# Autodesk Inventor assembly: sparIntermediateFlat_US
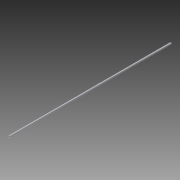
[picture p0: Inventor's stored thumbnail of the model, 180x180]
Saved by Autodesk Inventor 2014 (Build 180170000, 170)
## iProperties
Created: 2015-03-27
Part Number: sparIntermediateFlat_US
Document SubType Name: Assembly
Designer: ddeboer
Author: ddeboer
## Documents named in this file (4)
- C:\Users\ddeboer\Desktop\hera-cad\surface\sparIntermediateFlat_US.iam
- C:\Users\ddeboer\Desktop\hera-cad\surface\pvcSection_2in.ipt
- C:\Users\ddeboer\Desktop\hera-cad\smallParts\coupler_2in.ipt
- C:\Users\ddeboer\Desktop\hera-cad\surface\pvcSection_2in_cut4intermed.ipt
## Components (3 placed, 3 different names)
1. pvcSection_2in:1 — Insert:1
2. coupler_2in:1 — Insert:1, Insert:2
3. pvcSection_2in_cut4intermed:1 — Insert:2
## Relationships (2: Insert 2)
- Insert:1 (-29.3624 mm): pvcSection_2in:1 ↔ coupler_2in:1
- Insert:2 (-29.3624 mm): coupler_2in:1 ↔ pvcSection_2in_cut4intermed:1
